# Autodesk Inventor assembly: Motor
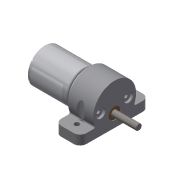
[picture p0: Inventor's stored thumbnail of the model, 180x180]
Saved by Autodesk Inventor 2018 (Build 220112000, 112)
## iProperties
Created: 2017-12-18
Part Number: Motor
Document SubType Name: Assembly
Designer: dsayers
Author: dsayers
## Documents named in this file (3)
- C:\Fun Projects\FTC\Motor.iam
- C:\Fun Projects\FTC\39530_txm-dc gearhead motor.ipt
- C:\Fun Projects\FTC\Motor Mount.ipt
## Components (2 placed, 2 different names)
1. 39530_txm-dc gearhead motor:1 — Flush:1, Flush:2
2. Motor Mount:1 — Flush:1, Flush:2
## Relationships (2: Flush 2)
- Flush:1: 39530_txm-dc gearhead motor:1 ↔ Motor Mount:1
- Flush:2: 39530_txm-dc gearhead motor:1 ↔ Motor Mount:1
